# Autodesk Inventor assembly: Sestava1
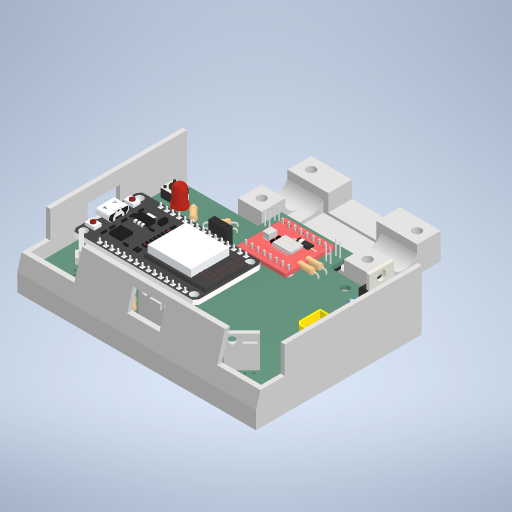
[picture p0: Inventor's stored thumbnail of the model, 512x512]
Saved by Autodesk Inventor 2024 (Build 280153000, 153)
## iProperties
Created: 2023-09-07
Part Number: Sestava1
Document SubType Name: Assembly
Designer: Simak
Author: Simak
## Documents named in this file (3)
- C:\Users\Simak\OneDrive\Dokumenty\GitHub\RoboCop\- 3D -\wip\Sestava1.iam
- C:\Users\Simak\OneDrive\Dokumenty\GitHub\RoboCop\- 3D -\wip\Součást1.ipt
- C:\Users\Simak\OneDrive\Dokumenty\GitHub\RoboCop\- PCB -\SUMEC THT\sumec\sumec.ipt
## Components (2 placed, 2 different names)
1. Součást1:1 — Vložit:1, Vložit:2
2. sumec:1 — Vložit:1, Vložit:2
## Relationships (2: Insert 2)
- Vložit:1 [Insert]: Součást1:1 ↔ sumec:1
- Vložit:2 [Insert]: Součást1:1 ↔ sumec:1
